# Autodesk Inventor assembly: Assembly_Opentrons_Autofocus_v2
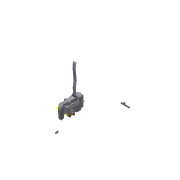
[picture p0: Inventor's stored thumbnail of the model, 180x180]
Saved by Autodesk Inventor 2019.4 (Build 234330000, 330)
## iProperties
Created: 2020-10-23
Part Number: Assembly_Opentrons_Autofocus_v2
Document SubType Name: Assembly
Designer: diederichbenedict
Author: diederichbenedict
## Documents named in this file (18)
- C:\Users\diederichbenedict\Dropbox\Dokumente\Promotion\PROJECTS\OPENTRONS\INVENTOR\Assembly_Opentrons_Autofocus_v2.iam
- C:\Users\diederichbenedict\Dropbox\Dokumente\Promotion\PROJECTS\OPENTRONS\INVENTOR\00_RasPi_Camera.ipt
- C:\Users\diederichbenedict\Dropbox\Dokumente\Promotion\PROJECTS\OPENTRONS\INVENTOR\00_spindel_slide.ipt
- C:\Users\diederichbenedict\Dropbox\Dokumente\Promotion\PROJECTS\OPENTRONS\INVENTOR\00_opticalpath.ipt
- C:\Users\diederichbenedict\Dropbox\Dokumente\Promotion\PROJECTS\OPENTRONS\INVENTOR\00_COMAR_Mirror_10mm.ipt
- C:\Users\diederichbenedict\Dropbox\Dokumente\Promotion\PROJECTS\OPENTRONS\INVENTOR\00_NEMA11.iam
- C:\Users\diederichbenedict\Dropbox\Dokumente\Promotion\PROJECTS\OPENTRONS\INVENTOR\00_objectivelens_10x.ipt
- C:\Users\diederichbenedict\Dropbox\Dokumente\Promotion\PROJECTS\OPENTRONS\INVENTOR\01_Slide_camera_v1.ipt
- C:\Users\diederichbenedict\Dropbox\Dokumente\Promotion\PROJECTS\OPENTRONS\INVENTOR\01_opticsmodule.ipt
- C:\Users\diederichbenedict\Dropbox\Dokumente\Promotion\PROJECTS\OPENTRONS\INVENTOR\01_Slide_camera_flexure_v1.ipt
- C:\Users\diederichbenedict\Documents\Inventor\Content Center Files\R2019\en-US\DIN 912\DIN 912 - M4 x 0.7 x 20 x 18.25.ipt
- C:\Users\diederichbenedict\Dropbox\Dokumente\Promotion\PROJECTS\OPENTRONS\INVENTOR\opentrons_gear2.ipt
- C:\Users\diederichbenedict\Dropbox\Dokumente\Promotion\PROJECTS\OPENTRONS\INVENTOR\opentrons_gear1.ipt
- C:\Users\diederichbenedict\Dropbox\Dokumente\Promotion\PROJECTS\OPENTRONS\INVENTOR\opentrons_Gearbox.ipt
- C:\Users\diederichbenedict\Dropbox\Dokumente\Promotion\PROJECTS\OPENTRONS\INVENTOR\00_MGN12H, LINEAR GUIDE BLOCK.ipt
- C:\Users\diederichbenedict\Dropbox\Dokumente\Promotion\PROJECTS\OPENTRONS\INVENTOR\STL\00_gear_rack.ipt
- C:\Users\diederichbenedict\Dropbox\Dokumente\Promotion\PROJECTS\OPENTRONS\INVENTOR\STL\00_gear_nema.ipt
- C:\Users\diederichbenedict\Dropbox\Dokumente\Promotion\PROJECTS\OPENTRONS\INVENTOR\00_LED_neopixel_single.ipt
## Components (17 placed, 17 different names)
1. 00_opticalpath:1 — Insert:9, Insert:11, Insert:12
2. 00_COMAR_Mirror_10mm:1 — Insert:11
3. 00_RasPi_Camera:1 — Insert:12, Angle:2
4. 00_MGN12H, LINEAR GUIDE BLOCK:1 — Angle:3
5. 00_spindel_slide:1
6. 00_NEMA11:2 [sub-assembly]
7. 00_objectivelens_10x:1 — Insert:9, Insert:16, Angle:3
8. 01_Slide_camera_v1:1 — Mate:3, Flush:12, Flush:13, Insert:14, Mate:4
9. 01_Slide_camera_flexure_v1:1 — Mate:3, Flush:12, Flush:13, Mate:5, Mate:6
10. Spur Gear2:1 — Insert:15
11. Spur Gear1:1 — Insert:14
12. DIN 912 - replaced by DIN EN ISO 4762 M4 x 20:1 — Insert:15, Mate:4
13. opentrons_Gearbox:1
14. 01_opticsmodule:1 — Insert:16, Mate:5, Mate:6
15. 00_gear_nema:1
16. 00_gear_rack:1
17. 00_LED_neopixel_single:1
## Relationships (18: Insert 6, Mate 5, Flush 5, Angle 2)
- [Mate]: 00_MGN12H, LINEAR GUIDE BLOCK:1 ↔ 00_NEMA11:2
- [Flush]: 00_MGN12H, LINEAR GUIDE BLOCK:1 ↔ 00_objectivelens_10x:1
- Insert:9: 00_opticalpath:1 ↔ 00_objectivelens_10x:1
- Insert:11: 00_opticalpath:1 ↔ 00_COMAR_Mirror_10mm:1
- Insert:12: 00_opticalpath:1 ↔ 00_RasPi_Camera:1
- Angle:2 (0 deg): 00_RasPi_Camera:1
- Mate:3: 01_Slide_camera_v1:1 ↔ 01_Slide_camera_flexure_v1:1
- Flush:12: 01_Slide_camera_v1:1 ↔ 01_Slide_camera_flexure_v1:1
- Flush:13: 01_Slide_camera_v1:1 ↔ 01_Slide_camera_flexure_v1:1
- Insert:14: 01_Slide_camera_v1:1 ↔ Spur Gear1:1
- Insert:15: Spur Gear2:1 ↔ DIN 912 - replaced by DIN EN ISO 4762 M4 x 20:1
- Mate:4: 01_Slide_camera_v1:1 ↔ DIN 912 - replaced by DIN EN ISO 4762 M4 x 20:1
- Insert:16: 00_objectivelens_10x:1 ↔ 01_opticsmodule:1
- [Flush]: 00_gear_nema:1 ↔ 00_gear_rack:1
- [Flush]: 00_gear_nema:1 ↔ 00_gear_rack:1
- Mate:5: 01_Slide_camera_flexure_v1:1 ↔ 01_opticsmodule:1
- Mate:6: 01_Slide_camera_flexure_v1:1 ↔ 01_opticsmodule:1
- Angle:3 (0 deg): 00_MGN12H, LINEAR GUIDE BLOCK:1 ↔ 00_objectivelens_10x:1
